# Autodesk Inventor assembly: DoubleCardan
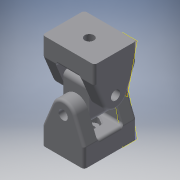
[picture p0: Inventor's stored thumbnail of the model, 180x180]
Saved by Autodesk Inventor 2018 (Build 220112000, 112)
## iProperties
Created: 2020-03-23
Part Number: DoubleCardan
Document SubType Name: Assembly
Designer: technik
Author: technik
## Documents named in this file (3)
- E:\repos-f\astro\ranger\cad\DoubleCardan.iam
- E:\repos-f\astro\ranger\cad\CardanHinge.ipt
- E:\repos-f\astro\ranger\cad\CardanJoint.ipt
## Components (3 placed, 2 different names)
1. CardanHinge:1 — Mate:2, Mate:3, Mate:4
2. CardanJoint:1 — Mate:3, Mate:4, Mate:5, Mate:6
3. CardanHinge:2 — Mate:5, Mate:6
## Relationships (5: Mate 5)
- Mate:2: CardanHinge:1
- Mate:3: CardanHinge:1 ↔ CardanJoint:1
- Mate:4: CardanHinge:1 ↔ CardanJoint:1
- Mate:5: CardanJoint:1 ↔ CardanHinge:2
- Mate:6: CardanJoint:1 ↔ CardanHinge:2
